# Autodesk Inventor assembly: CIM-Sim
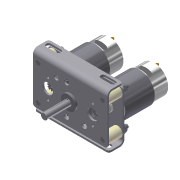
[picture p0: Inventor's stored thumbnail of the model, 180x180]
Saved by Autodesk Inventor 2011 (Build 150239000, 239)
## iProperties
Created: 2012-06-04
Part Number: CIM-Sim
Document SubType Name: Assembly
Designer: Nemo
Author: Nemo
## Documents named in this file (12)
- H:\Nemo\Documents\Robotics\COTS Parts\Gearboxes\CIM-Sim.iam
- H:\Nemo\Documents\Robotics\COTS Parts\Gearboxes\Housings\CIM-Sim Plate.ipt
- H:\Nemo\Documents\Robotics\COTS Parts\Gearboxes\Housings\CIM-Sim Plate Spacer.ipt
- H:\Nemo\Documents\Robotics\COTS Parts\Gearboxes\Bearings\Bearing F698ZZ.ipt
- H:\Nemo\Documents\Robotics\COTS Parts\Gearboxes\Shafts\CIM-Sim Shaft.ipt
- H:\Nemo\Documents\Robotics\COTS Parts\Gearboxes\Gears\Gear 32dp 375hex 60T.ipt
- H:\Nemo\Documents\Robotics\COTS Parts\Gearboxes\Spacers\CIM-Sim Spacer 177x500.ipt
- H:\Nemo\Documents\Robotics\COTS Parts\Fasteners\10-32 PEM-Stud.ipt
- H:\Nemo\Documents\Robotics\COTS Parts\Fasteners\10-32 locknut.ipt
- H:\Nemo\Documents\Robotics\COTS Parts\Motors\Motors_BaneBots_RS-550.ipt
- H:\Nemo\Documents\Robotics\COTS Parts\Fasteners\4-40 SHCS x500.ipt
- H:\Nemo\Documents\Robotics\COTS Parts\Gearboxes\Gears\Gear 32dp 125press 12T.ipt
## Components (27 placed, 11 different names)
1. CIM-Sim Plate:1 — Mate:1, Mate:2, Insert:1, Insert:2, Insert:3, Insert:4, Mate:4, Insert:5, Insert:8, Insert:9, Insert:10, Insert:11, Angle:2, Angle:3
2. CIM-Sim Plate:2 — Mate:1, Mate:2, Mate:3, Insert:6, Insert:12, Insert:13, Insert:14, Insert:15, Mate:9, Insert:16, Insert:17, Insert:18, Insert:19, Insert:20, Insert:21
3. CIM-Sim Plate Spacer:1 — Insert:2
4. CIM-Sim Plate Spacer:2 — Insert:1
5. CIM-Sim Plate Spacer:3 — Insert:3
6. CIM-Sim Plate Spacer:4 — Insert:4, Mate:3
7. Bearing F698ZZ:1 — Insert:5, Mate:8
8. Bearing F698ZZ:2 — Insert:6, Insert:7, Mate:7
9. CIM-Sim Shaft:1 — Mate:4, Insert:7, Mate:5, Mate:6, Angle:1
10. Gear 60T 32dp 375hex:1 — Mate:5, Angle:1, Mate:8, Flush:1, Flush:2
11. CIM-Sim Spacer 177x500:1 — Mate:6, Mate:7
12. 10-32 PEM-Stud:1 — Insert:10
13. 10-32 PEM-Stud:2 — Insert:11
14. 10-32 PEM-Stud:3 — Insert:9
15. 10-32 PEM-Stud:4 — Insert:8
16. 10-32 locknut:1 — Insert:12
17. 10-32 locknut:2 — Insert:13
18. 10-32 locknut:3 — Insert:14
19. 10-32 locknut:4 — Insert:15
20. Motors_BaneBots_RS-550:1 — Insert:17, Angle:3, Mate:11
21. Motors_BaneBots_RS-550:2 — Mate:9, Insert:16, Angle:2, Mate:10
22. 4-40 SHCS x500:1 — Insert:21
23. 4-40 SHCS x500:2 — Insert:20
24. 4-40 SHCS x500:3 — Insert:19
25. 4-40 SHCS x500:4 — Insert:18
26. Gear 12T 32dp 125press:1 — Mate:11, Flush:1
27. Gear 12T 32dp 125press:2 — Mate:10, Flush:2
## Relationships (37: Insert 21, Mate 11, Angle 3, Flush 2)
- Mate:1: CIM-Sim Plate:1 ↔ CIM-Sim Plate:2
- Mate:2: CIM-Sim Plate:1 ↔ CIM-Sim Plate:2
- Insert:1: CIM-Sim Plate:1 ↔ CIM-Sim Plate Spacer:2
- Insert:2: CIM-Sim Plate:1 ↔ CIM-Sim Plate Spacer:1
- Insert:3: CIM-Sim Plate:1 ↔ CIM-Sim Plate Spacer:3
- Insert:4: CIM-Sim Plate:1 ↔ CIM-Sim Plate Spacer:4
- Mate:3: CIM-Sim Plate:2 ↔ CIM-Sim Plate Spacer:4
- Mate:4: CIM-Sim Plate:1 ↔ CIM-Sim Shaft:1
- Insert:5: CIM-Sim Plate:1 ↔ Bearing F698ZZ:1
- Insert:6: CIM-Sim Plate:2 ↔ Bearing F698ZZ:2
- Insert:7: Bearing F698ZZ:2 ↔ CIM-Sim Shaft:1
- Mate:5: CIM-Sim Shaft:1 ↔ Gear 60T 32dp 375hex:1
- Mate:6: CIM-Sim Shaft:1 ↔ CIM-Sim Spacer 177x500:1
- Mate:7: Bearing F698ZZ:2 ↔ CIM-Sim Spacer 177x500:1
- Angle:1 (0 deg): CIM-Sim Shaft:1 ↔ Gear 60T 32dp 375hex:1
- Mate:8: Bearing F698ZZ:1 ↔ Gear 60T 32dp 375hex:1
- Insert:8: CIM-Sim Plate:1 ↔ 10-32 PEM-Stud:4
- Insert:9: CIM-Sim Plate:1 ↔ 10-32 PEM-Stud:3
- Insert:10: CIM-Sim Plate:1 ↔ 10-32 PEM-Stud:1
- Insert:11: CIM-Sim Plate:1 ↔ 10-32 PEM-Stud:2
- Insert:12: CIM-Sim Plate:2 ↔ 10-32 locknut:1
- Insert:13: CIM-Sim Plate:2 ↔ 10-32 locknut:2
- Insert:14: CIM-Sim Plate:2 ↔ 10-32 locknut:3
- Insert:15: CIM-Sim Plate:2 ↔ 10-32 locknut:4
- Mate:9: CIM-Sim Plate:2 ↔ Motors_BaneBots_RS-550:2
- Insert:16: CIM-Sim Plate:2 ↔ Motors_BaneBots_RS-550:2
- Angle:2 (0 deg): CIM-Sim Plate:1 ↔ Motors_BaneBots_RS-550:2
- Insert:17: CIM-Sim Plate:2 ↔ Motors_BaneBots_RS-550:1
- Angle:3 (0 deg): CIM-Sim Plate:1 ↔ Motors_BaneBots_RS-550:1
- Insert:18: CIM-Sim Plate:2 ↔ 4-40 SHCS x500:4
- Insert:19: CIM-Sim Plate:2 ↔ 4-40 SHCS x500:3
- Insert:20: CIM-Sim Plate:2 ↔ 4-40 SHCS x500:2
- Insert:21: CIM-Sim Plate:2 ↔ 4-40 SHCS x500:1
- Mate:10: Motors_BaneBots_RS-550:2 ↔ Gear 12T 32dp 125press:2
- Mate:11: Motors_BaneBots_RS-550:1 ↔ Gear 12T 32dp 125press:1
- Flush:1: Gear 60T 32dp 375hex:1 ↔ Gear 12T 32dp 125press:1
- Flush:2: Gear 60T 32dp 375hex:1 ↔ Gear 12T 32dp 125press:2
